# Autodesk Inventor assembly: FRC200-1
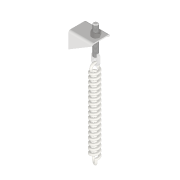
[picture p0: Inventor's stored thumbnail of the model, 180x180]
Saved by Autodesk Inventor 2020 (Build 240168000, 168)
## iProperties
Created: 2020-02-19
Part Number: FRC200-1
Document SubType Name: Assembly
Designer: Juan Carlos Botero
Mass: 373.254 g
Surface Area: 498.375 cm^2
Volume: 97.5899 cm^3
Density: 3.82472 g/cm^3
Author: Juan Carlos Botero
Title: SOPORTE AJUSTABLE
## Documents named in this file (5)
- D:\Drives\OneDrive\Carlos_2\02 TRABAJOS\MULTIPLO\Conveyor\ENSAMBLE - Copy\Tensor_.iam
- D:\Drives\OneDrive\Carlos_2\02 TRABAJOS\MULTIPLO\Conveyor\ENSAMBLE - Copy\Break_Tensor.ipt
- D:\Drives\OneDrive\Carlos_2\02 TRABAJOS\MULTIPLO\Conveyor\ENSAMBLE\Eje delantero _1_\Design Accelerator\Extension Spring2.iam
- C:\Users\Charlie\Documents\Inventor\Content Center Files\R2020\en-US\AS 2465(1)\AS 2465 - 1_2  UNC(1).ipt
- D:\Drives\OneDrive\Carlos_2\02 TRABAJOS\MULTIPLO\Conveyor\ENSAMBLE - Copy\Soporte Fijo.ipt
## Components (4 placed, 4 different names)
1. Break_Tensor:1 — Angle:1, Mate:3, Tangent:1, Mate:5
2. Extension Spring:1 [sub-assembly] — Mate:2, Tangent:1
3. AS 2465 - Inch 1/2  UNC:1
4. Soporte Fijo:1 — Mate:5
## Relationships (5: Mate 3, Angle 1, Tangent 1)
- Mate:2: Extension Spring:1
- Angle:1 (90 deg): Break_Tensor:1
- Mate:3: Break_Tensor:1
- Tangent:1: Break_Tensor:1 ↔ Extension Spring:1
- Mate:5: Break_Tensor:1 ↔ Soporte Fijo:1
